# Autodesk Inventor assembly: CLAW
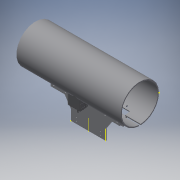
[picture p0: Inventor's stored thumbnail of the model, 180x180]
Saved by Autodesk Inventor 2017 (Build 210142000, 142)
## iProperties
Created: 2017-04-09
Part Number: CLAW
Document SubType Name: Assembly
Designer: s4461999
Author: s4461999
## Documents named in this file (6)
- U:\CAD\CLAW.iam
- U:\CAD\lowerClaw.ipt
- U:\CAD\upperClaw.ipt
- U:\CAD\adjustmentHingePlate.ipt
- U:\CAD\plate.ipt
- \\puffball.labs.eait.uq.edu.au\s4461999\Desktop\TOWER PRO MG-995, ANALOG SERVO.iam
## Components (17 placed, 5 different names)
1. adjustmentHingePlate:1 — Mate:11, Mate:12, Flush:2, Flush:9
2. adjustmentHingePlate:2 — Mate:12, Flush:2
3. adjustmentHingePlate:3 — Mate:13, Mate:14, Mate:20, Mate:23, Mate:25, Mate:29, Mate:31, Mate:34, Mate:35, Mate:36, Flush:11, Flush:12
4. adjustmentHingePlate:4 — Mate:14, Mate:15, Mate:19, Mate:20, Mate:24, Mate:28, Mate:29, Mate:30, Mate:31, Mate:36, Mate:37, Flush:10, Flush:11
5. adjustmentHingePlate:5 — Mate:15, Mate:19, Mate:24, Mate:28, Mate:30, Flush:10
6. adjustmentHingePlate:6 — Mate:9, Flush:4, Flush:5
7. adjustmentHingePlate:7 — Mate:8, Mate:9, Flush:5, Flush:6
8. adjustmentHingePlate:8 — Mate:7, Mate:8, Flush:3, Flush:6, Flush:7
9. adjustmentHingePlate:9 — Mate:6, Mate:22, Mate:27, Mate:32, Flush:14
10. adjustmentHingePlate:10 — Mate:5, Mate:6, Mate:21, Mate:22, Mate:26, Mate:27, Mate:32, Mate:33, Mate:37, Flush:13, Flush:14
11. adjustmentHingePlate:11 — Mate:10, Mate:11, Flush:1, Flush:3, Flush:4, Flush:8, Flush:9
12. adjustmentHingePlate:12 — Mate:4, Mate:5, Mate:21, Mate:23, Mate:25, Mate:26, Mate:33, Mate:34, Mate:35, Flush:13
13. plate:1 — Mate:4, Mate:7, Mate:10, Mate:13, Flush:1, Flush:7, Flush:8, Flush:12, Mate:38, Mate:39
14. TOWER PRO MG-995, ANALOG SERVO:1 [sub-assembly] — Mate:39, Flush:15, Flush:16, Flush:17
15. TOWER PRO MG-995, ANALOG SERVO:2 [sub-assembly] — Mate:38, Flush:15, Flush:16, Flush:17
16. lowerClaw:1 — Mate:40, Flush:18, Mate:41
17. upperClaw:1 — Mate:40, Flush:18, Mate:41
## Relationships (53: Mate 35, Flush 18)
- Mate:4: adjustmentHingePlate:12 ↔ plate:1
- Mate:5: adjustmentHingePlate:10 ↔ adjustmentHingePlate:12
- Mate:6: adjustmentHingePlate:9 ↔ adjustmentHingePlate:10
- Mate:7: adjustmentHingePlate:8 ↔ plate:1
- Mate:8: adjustmentHingePlate:7 ↔ adjustmentHingePlate:8
- Mate:9: adjustmentHingePlate:6 ↔ adjustmentHingePlate:7
- Mate:10: adjustmentHingePlate:11 ↔ plate:1
- Mate:11: adjustmentHingePlate:1 ↔ adjustmentHingePlate:11
- Mate:12: adjustmentHingePlate:1 ↔ adjustmentHingePlate:2
- Mate:13: adjustmentHingePlate:3 ↔ plate:1
- Mate:14: adjustmentHingePlate:3 ↔ adjustmentHingePlate:4
- Mate:15: adjustmentHingePlate:4 ↔ adjustmentHingePlate:5
- Mate:19: adjustmentHingePlate:4 ↔ adjustmentHingePlate:5
- Mate:20: adjustmentHingePlate:3 ↔ adjustmentHingePlate:4
- Mate:21: adjustmentHingePlate:10 ↔ adjustmentHingePlate:12
- Mate:22: adjustmentHingePlate:9 ↔ adjustmentHingePlate:10
- Mate:23: adjustmentHingePlate:3 ↔ adjustmentHingePlate:12
- Mate:24: adjustmentHingePlate:4 ↔ adjustmentHingePlate:5
- Mate:25: adjustmentHingePlate:3 ↔ adjustmentHingePlate:12
- Mate:26: adjustmentHingePlate:10 ↔ adjustmentHingePlate:12
- Mate:27: adjustmentHingePlate:9 ↔ adjustmentHingePlate:10
- Mate:28: adjustmentHingePlate:4 ↔ adjustmentHingePlate:5
- Mate:29: adjustmentHingePlate:3 ↔ adjustmentHingePlate:4
- Mate:30: adjustmentHingePlate:4 ↔ adjustmentHingePlate:5
- Mate:31: adjustmentHingePlate:3 ↔ adjustmentHingePlate:4
- Mate:32: adjustmentHingePlate:9 ↔ adjustmentHingePlate:10
- Mate:33: adjustmentHingePlate:10 ↔ adjustmentHingePlate:12
- Mate:34: adjustmentHingePlate:3 ↔ adjustmentHingePlate:12
- Mate:35: adjustmentHingePlate:3 ↔ adjustmentHingePlate:12
- Mate:36: adjustmentHingePlate:3 ↔ adjustmentHingePlate:4
- Mate:37: adjustmentHingePlate:4 ↔ adjustmentHingePlate:10
- Flush:1: adjustmentHingePlate:11 ↔ plate:1
- Flush:2: adjustmentHingePlate:1 ↔ adjustmentHingePlate:2
- Flush:3: adjustmentHingePlate:8 ↔ adjustmentHingePlate:11
- Flush:4: adjustmentHingePlate:6 ↔ adjustmentHingePlate:11
- Flush:5: adjustmentHingePlate:6 ↔ adjustmentHingePlate:7
- Flush:6: adjustmentHingePlate:7 ↔ adjustmentHingePlate:8
- Flush:7: adjustmentHingePlate:8 ↔ plate:1
- Flush:8: adjustmentHingePlate:11 ↔ plate:1
- Flush:9: adjustmentHingePlate:1 ↔ adjustmentHingePlate:11
- Flush:10: adjustmentHingePlate:4 ↔ adjustmentHingePlate:5
- Flush:11: adjustmentHingePlate:3 ↔ adjustmentHingePlate:4
- Flush:12: adjustmentHingePlate:3 ↔ plate:1
- Flush:13: adjustmentHingePlate:10 ↔ adjustmentHingePlate:12
- Flush:14: adjustmentHingePlate:9 ↔ adjustmentHingePlate:10
- Mate:38: plate:1 ↔ TOWER PRO MG-995, ANALOG SERVO:2
- Mate:39: plate:1 ↔ TOWER PRO MG-995, ANALOG SERVO:1
- Flush:15: TOWER PRO MG-995, ANALOG SERVO:1 ↔ TOWER PRO MG-995, ANALOG SERVO:2
- Flush:16: TOWER PRO MG-995, ANALOG SERVO:1 ↔ TOWER PRO MG-995, ANALOG SERVO:2
- Flush:17: TOWER PRO MG-995, ANALOG SERVO:1 ↔ TOWER PRO MG-995, ANALOG SERVO:2
- Mate:40: lowerClaw:1 ↔ upperClaw:1
- Flush:18: lowerClaw:1 ↔ upperClaw:1
- Mate:41: lowerClaw:1 ↔ upperClaw:1
